# Autodesk Inventor assembly: 0_Entire_Assembly
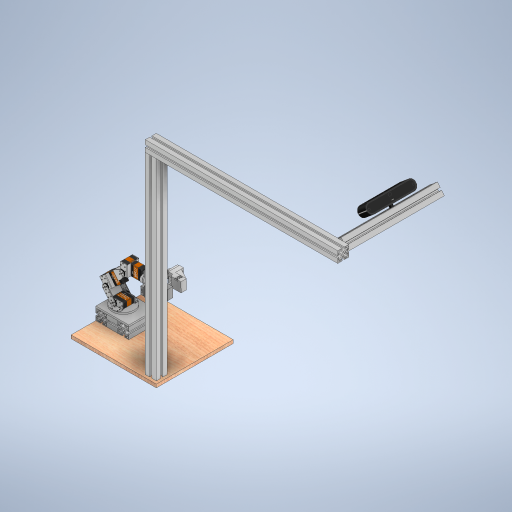
[picture p0: Inventor's stored thumbnail of the model, 512x512]
Saved by Autodesk Inventor 2024 (Build 280153000, 153)
## iProperties
Created: 2023-08-24
Part Number: 0_Entire_Assembly
Document SubType Name: Assembly
Designer: chanh
Author: chanh
## Documents named in this file (4)
- C:\Users\박동준\OneDrive - 연세대학교 (Yonsei University)\바탕 화면\박동준\대학생할\로봇\Humanoid\6축 매니퓰레이터\하드웨어\rh_plus_7_axis_robot_arm_hardware\Assembly\0_Entire_Assembly.iam
- C:\Users\박동준\OneDrive - 연세대학교 (Yonsei University)\바탕 화면\박동준\대학생할\로봇\Humanoid\6축 매니퓰레이터\하드웨어\rh_plus_7_axis_robot_arm_hardware\Assembly\2_Arm.iam
- C:\Users\박동준\OneDrive - 연세대학교 (Yonsei University)\바탕 화면\박동준\대학생할\로봇\Humanoid\6축 매니퓰레이터\하드웨어\rh_plus_7_axis_robot_arm_hardware\Assembly\3_Gripper.iam
- C:\Users\박동준\OneDrive - 연세대학교 (Yonsei University)\바탕 화면\박동준\대학생할\로봇\Humanoid\6축 매니퓰레이터\하드웨어\rh_plus_7_axis_robot_arm_hardware\Assembly\1_Base.iam
## Components (3 placed, 3 different names)
1. 1_Base:1 [sub-assembly] — Rigid:2
2. 2_Arm:1 [sub-assembly] — Flush:1, Flush:2, Flush:3, Rigid:1, Rigid:2
3. 3_Gripper:1 [sub-assembly] — Rigid:1
## Relationships (5: Flush 3, WeldJoint 2)
- Flush:1: 2_Arm:1
- Flush:2: 2_Arm:1
- Flush:3: 2_Arm:1
- Rigid:1 [WeldJoint]: 2_Arm:1 ↔ 3_Gripper:1
- Rigid:2 [WeldJoint]: 1_Base:1 ↔ 2_Arm:1
